# Autodesk Inventor assembly: battery_box_24V
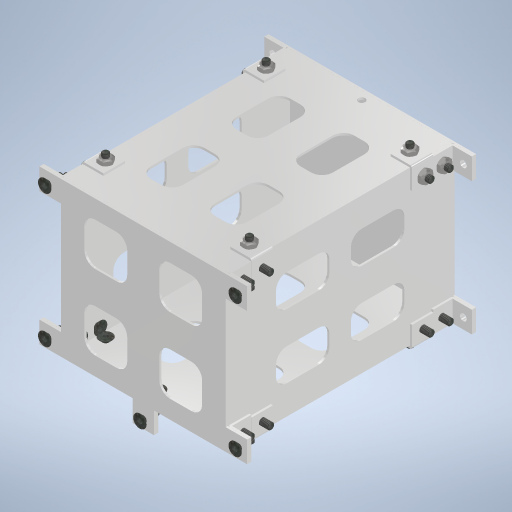
[picture p0: Inventor's stored thumbnail of the model, 512x512]
Saved by Autodesk Inventor 2023 (Build 270158000, 158)
## iProperties
Created: 2023-05-28
Part Number: battery_box_24V
Document SubType Name: Assembly
Designer: 310611102
Author: 310611102
## Documents named in this file (9)
- C:\Users\310611102\Documents\Inventor\SSR\avionics_2023ver\electronics\battery box\battery_box_ver3\battery_box_24V.iam
- C:\Users\310611102\Documents\Inventor\SSR\avionics_2023ver\electronics\battery box\battery_box_ver3\battery_box_24V_base.ipt
- C:\Users\310611102\Documents\Inventor\SSR\avionics_2023ver\electronics\battery box\battery_box_ver3\battery_box_24V_side1.ipt
- C:\Users\310611102\Documents\Inventor\SSR\avionics_2023ver\electronics\battery box\battery_box_ver3\connector.ipt
- C:\Users\310611102\Documents\Inventor\SSR\avionics_2023ver\electronics\battery box\battery_box_ver3\battery_box_24V_front.ipt
- C:\Users\310611102\Documents\Inventor\SSR\avionics_2023ver\electronics\battery box\battery_box_ver3\battery_box_24V_back.ipt
- C:\Users\310611102\Documents\Inventor\SSR\avionics_2023ver\electronics\battery box\battery_box_ver3\battery_box_24V_top.ipt
- C:\Users\310611102\Documents\Inventor\SSR\avionics_2023ver\electronics\ISO 4032 - M3 - ISO.ipt
- C:\Users\310611102\Documents\Inventor\SSR\avionics_2023ver\electronics\ISO 10642 - M3 x  8.ipt
## Components (66 placed, 8 different names)
1. battery_box_24V_base:1 — Insert:1, Insert:3, Insert:14, Insert:15, Mate:2, Flush:2, Insert:22, Mate:3, Flush:5
2. battery_box_24V_side1:1 — Insert:21, Insert:23, Cylindrical:15, Cylindrical:17, Insert:26, Insert:30, Cylindrical:18, Cylindrical:24, Insert:43, Insert:45, Insert:50, Insert:51, Insert:68, Insert:69, Insert:72, Insert:73
3. connector:1 — Insert:1, Insert:21, Insert:75
4. connector:2 — Insert:34, Insert:38
5. connector:3 — Insert:3, Insert:17, Insert:78
6. connector:4 — Insert:26, Insert:41
7. battery_box_24V_side1:2 — Insert:16, Insert:17, Cylindrical:9, Cylindrical:13, Insert:27, Insert:34, Cylindrical:20, Cylindrical:25, Insert:47, Insert:48, Insert:55, Insert:56, Insert:57, Insert:58, Insert:60, Insert:61
8. battery_box_24V_front:1 — Mate:2, Flush:2, Cylindrical:12, Cylindrical:14, Insert:36, Cylindrical:19, Cylindrical:21, Insert:59, Insert:62, Insert:63, Insert:64, Insert:70, Insert:71
9. connector:5 — Insert:27, Insert:39, Insert:81, Insert:83
10. connector:7 — Cylindrical:9, Insert:76, Insert:77
11. connector:8 — Cylindrical:12, Cylindrical:13
12. connector:9 — Insert:37
13. connector:10 — Cylindrical:14, Cylindrical:15
14. connector:11 — Insert:30, Insert:40
15. connector:13 — Insert:14, Insert:16
16. connector:14 — Insert:15, Insert:36
17. connector:16 — Insert:22, Insert:23
18. connector:17 — Cylindrical:17, Insert:44, Insert:74
19. connector:18 — Cylindrical:18, Cylindrical:19
20. connector:19 — Cylindrical:25, Cylindrical:26, Insert:80, Insert:82
21. connector:20 — Cylindrical:23, Cylindrical:24, Insert:79
22. connector:21 — Cylindrical:20, Cylindrical:21
23. battery_box_24V_back:1 — Mate:3, Flush:5, Cylindrical:23, Cylindrical:26, Insert:42, Insert:46, Insert:49, Insert:52
24. battery_box_24V_top:1 — Insert:37, Insert:38, Insert:39, Insert:40, Insert:41, Insert:53, Insert:54, Insert:65, Insert:66, Insert:67
25. ISO 10642 M3x8:1 — Insert:42
26. ISO 10642 M3x8:2 — Insert:43
27. ISO 10642 M3x8:3 — Insert:45
28. ISO 10642 M3x8:4 — Insert:46
29. ISO 10642 M3x8:5 — Insert:47
30. ISO 10642 M3x8:6 — Insert:48
31. ISO 10642 M3x8:7 — Insert:49
32. ISO 10642 M3x8:8 — Insert:50
33. ISO 10642 M3x8:9 — Insert:51
34. ISO 10642 M3x8:10 — Insert:52
35. ISO 10642 M3x8:11 — Insert:53
36. ISO 10642 M3x8:12 — Insert:54
37. ISO 10642 M3x8:13 — Insert:55
38. ISO 10642 M3x8:14 — Insert:56
39. ISO 10642 M3x8:15 — Insert:57
40. ISO 10642 M3x8:16 — Insert:58
41. ISO 10642 M3x8:17 — Insert:59
42. ISO 10642 M3x8:18 — Insert:60
43. ISO 10642 M3x8:19 — Insert:61
44. ISO 10642 M3x8:20 — Insert:62
45. ISO 10642 M3x8:21 — Insert:63
46. ISO 10642 M3x8:22 — Insert:64
47. ISO 10642 M3x8:23 — Insert:65
48. ISO 10642 M3x8:24 — Insert:66
49. ISO 10642 M3x8:25 — Insert:67
50. ISO 10642 M3x8:26 — Insert:68
51. ISO 10642 M3x8:27 — Insert:69
52. ISO 10642 M3x8:28 — Insert:70
53. ISO 10642 M3x8:29 — Insert:71
54. ISO 10642 M3x8:30 — Insert:72
55. ISO 10642 M3x8:31 — Insert:73
56. ISO 4032 M3:1 — Insert:44
57. ISO 4032 M3:2 — Insert:74
58. ISO 4032 M3:3 — Insert:75
59. ISO 4032 M3:4 — Insert:76
60. ISO 4032 M3:5 — Insert:77
61. ISO 4032 M3:6 — Insert:78
62. ISO 4032 M3:7 — Insert:79
63. ISO 4032 M3:8 — Insert:80
64. ISO 4032 M3:9 — Insert:81
65. ISO 4032 M3:10 — Insert:82
66. ISO 4032 M3:11 — Insert:83
## Relationships (79: Insert 61, CylindricalJoint 14, Mate 2, Flush 2)
- Insert:1: battery_box_24V_base:1 ↔ connector:1
- Insert:3: battery_box_24V_base:1 ↔ connector:3
- Insert:14: battery_box_24V_base:1 ↔ connector:13
- Insert:15: battery_box_24V_base:1 ↔ connector:14
- Insert:16: battery_box_24V_side1:2 ↔ connector:13
- Insert:17: connector:3 ↔ battery_box_24V_side1:2
- Cylindrical:9: battery_box_24V_side1:2 ↔ connector:7
- Mate:2: battery_box_24V_base:1 ↔ battery_box_24V_front:1
- Flush:2: battery_box_24V_base:1 ↔ battery_box_24V_front:1
- Insert:21: battery_box_24V_side1:1 ↔ connector:1
- Insert:22: battery_box_24V_base:1 ↔ connector:16
- Insert:23: battery_box_24V_side1:1 ↔ connector:16
- Cylindrical:12: battery_box_24V_front:1 ↔ connector:8
- Cylindrical:13: battery_box_24V_side1:2 ↔ connector:8
- Cylindrical:14: battery_box_24V_front:1 ↔ connector:10
- Cylindrical:15: battery_box_24V_side1:1 ↔ connector:10
- Cylindrical:17: battery_box_24V_side1:1 ↔ connector:17
- Insert:26: battery_box_24V_side1:1 ↔ connector:4
- Insert:27: battery_box_24V_side1:2 ↔ connector:5
- Insert:30: battery_box_24V_side1:1 ↔ connector:11
- Insert:34: connector:2 ↔ battery_box_24V_side1:2
- Insert:36: battery_box_24V_front:1 ↔ connector:14
- Cylindrical:18: battery_box_24V_side1:1 ↔ connector:18
- Cylindrical:19: battery_box_24V_front:1 ↔ connector:18
- Cylindrical:20: battery_box_24V_side1:2 ↔ connector:21
- Cylindrical:21: battery_box_24V_front:1 ↔ connector:21
- Mate:3: battery_box_24V_base:1 ↔ battery_box_24V_back:1
- Flush:5: battery_box_24V_base:1 ↔ battery_box_24V_back:1
- Cylindrical:23: connector:20 ↔ battery_box_24V_back:1
- Cylindrical:24: battery_box_24V_side1:1 ↔ connector:20
- Cylindrical:25: battery_box_24V_side1:2 ↔ connector:19
- Cylindrical:26: connector:19 ↔ battery_box_24V_back:1
- Insert:37: connector:9 ↔ battery_box_24V_top:1
- Insert:38: connector:2 ↔ battery_box_24V_top:1
- Insert:39: connector:5 ↔ battery_box_24V_top:1
- Insert:40: connector:11 ↔ battery_box_24V_top:1
- Insert:41: connector:4 ↔ battery_box_24V_top:1
- Insert:42: battery_box_24V_back:1 ↔ ISO 10642 M3x8:1
- Insert:43: battery_box_24V_side1:1 ↔ ISO 10642 M3x8:2
- Insert:44: connector:17 ↔ ISO 4032 M3:1
- Insert:45: battery_box_24V_side1:1 ↔ ISO 10642 M3x8:3
- Insert:46: battery_box_24V_back:1 ↔ ISO 10642 M3x8:4
- Insert:47: battery_box_24V_side1:2 ↔ ISO 10642 M3x8:5
- Insert:48: battery_box_24V_side1:2 ↔ ISO 10642 M3x8:6
- Insert:49: battery_box_24V_back:1 ↔ ISO 10642 M3x8:7
- Insert:50: battery_box_24V_side1:1 ↔ ISO 10642 M3x8:8
- Insert:51: battery_box_24V_side1:1 ↔ ISO 10642 M3x8:9
- Insert:52: battery_box_24V_back:1 ↔ ISO 10642 M3x8:10
- Insert:53: battery_box_24V_top:1 ↔ ISO 10642 M3x8:11
- Insert:54: battery_box_24V_top:1 ↔ ISO 10642 M3x8:12
- Insert:55: battery_box_24V_side1:2 ↔ ISO 10642 M3x8:13
- Insert:56: battery_box_24V_side1:2 ↔ ISO 10642 M3x8:14
- Insert:57: battery_box_24V_side1:2 ↔ ISO 10642 M3x8:15
- Insert:58: battery_box_24V_side1:2 ↔ ISO 10642 M3x8:16
- Insert:59: battery_box_24V_front:1 ↔ ISO 10642 M3x8:17
- Insert:60: battery_box_24V_side1:2 ↔ ISO 10642 M3x8:18
- Insert:61: battery_box_24V_side1:2 ↔ ISO 10642 M3x8:19
- Insert:62: battery_box_24V_front:1 ↔ ISO 10642 M3x8:20
- Insert:63: battery_box_24V_front:1 ↔ ISO 10642 M3x8:21
- Insert:64: battery_box_24V_front:1 ↔ ISO 10642 M3x8:22
- Insert:65: battery_box_24V_top:1 ↔ ISO 10642 M3x8:23
- Insert:66: battery_box_24V_top:1 ↔ ISO 10642 M3x8:24
- Insert:67: battery_box_24V_top:1 ↔ ISO 10642 M3x8:25
- Insert:68: battery_box_24V_side1:1 ↔ ISO 10642 M3x8:26
- Insert:69: battery_box_24V_side1:1 ↔ ISO 10642 M3x8:27
- Insert:70: battery_box_24V_front:1 ↔ ISO 10642 M3x8:28
- Insert:71: battery_box_24V_front:1 ↔ ISO 10642 M3x8:29
- Insert:72: battery_box_24V_side1:1 ↔ ISO 10642 M3x8:30
- Insert:73: battery_box_24V_side1:1 ↔ ISO 10642 M3x8:31
- Insert:74: connector:17 ↔ ISO 4032 M3:2
- Insert:75: connector:1 ↔ ISO 4032 M3:3
- Insert:76: connector:7 ↔ ISO 4032 M3:4
- Insert:77: connector:7 ↔ ISO 4032 M3:5
- Insert:78: connector:3 ↔ ISO 4032 M3:6
- Insert:79: connector:20 ↔ ISO 4032 M3:7
- Insert:80: connector:19 ↔ ISO 4032 M3:8
- Insert:81: connector:5 ↔ ISO 4032 M3:9
- Insert:82: connector:19 ↔ ISO 4032 M3:10
- Insert:83: connector:5 ↔ ISO 4032 M3:11
